# Autodesk Inventor assembly: set1_to_print-july21
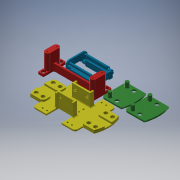
[picture p0: Inventor's stored thumbnail of the model, 180x180]
Saved by Autodesk Inventor 2017 SP1 (Build 210196100, 196)
## iProperties
Part Number: set1_to_print-july21
Material: Générique
Document SubType Name: Assembly
Designer: tmonglon
Author: tmonglon
## Documents named in this file (5)
- D:\Inventor\Ahmet\design-files-21jul2017\design-jul2017\design-modified\set1_to_print-july21.iam
- D:\Inventor\Ahmet\design-files-21jul2017\design-jul2017\design-modified\blue_part-july21.ipt
- D:\Inventor\Ahmet\design-files-21jul2017\design-jul2017\design-modified\red_part-july21.ipt
- D:\Inventor\Ahmet\design-files-21jul2017\design-jul2017\design-modified\green_part-july21.ipt
- D:\Inventor\Ahmet\design-files-21jul2017\design-jul2017\design-modified\yellow_part-july21.ipt
## Components (6 placed, 4 different names)
1. yellow_part-july21:1 — Placage:1, Affleurement:1, Affleurement:2, Affleurement:3, Affleurement:4, Affleurement:5, Placage:4, Placage:5, Placage:7
2. blue_part-july21:1 — Affleurement:5, Placage:2, Placage:3
3. blue_part-july21:2 — Affleurement:4, Placage:2, Placage:3, Placage:6
4. green_part-july21:1 — Affleurement:3, Affleurement:6, Placage:7
5. green_part-july21:2 — Affleurement:2, Affleurement:6
6. red_part-july21:1 — Affleurement:1, Placage:4, Placage:5, Placage:6
## Relationships (13: Mate 7, Flush 6)
- Placage:1 [Mate]: yellow_part-july21:1
- Affleurement:1 [Flush]: yellow_part-july21:1 ↔ red_part-july21:1
- Affleurement:2 [Flush]: yellow_part-july21:1 ↔ green_part-july21:2
- Affleurement:3 [Flush]: yellow_part-july21:1 ↔ green_part-july21:1
- Affleurement:4 [Flush]: yellow_part-july21:1 ↔ blue_part-july21:2
- Affleurement:5 [Flush]: yellow_part-july21:1 ↔ blue_part-july21:1
- Placage:2 [Mate] (2 mm): blue_part-july21:1 ↔ blue_part-july21:2
- Placage:3 [Mate] (42 mm): blue_part-july21:1 ↔ blue_part-july21:2
- Placage:4 [Mate] (2 mm): yellow_part-july21:1 ↔ red_part-july21:1
- Placage:5 [Mate] (8 mm): yellow_part-july21:1 ↔ red_part-july21:1
- Placage:6 [Mate] (2 mm): blue_part-july21:2 ↔ red_part-july21:1
- Affleurement:6 [Flush]: green_part-july21:1 ↔ green_part-july21:2
- Placage:7 [Mate] (3 mm): yellow_part-july21:1 ↔ green_part-july21:1
